# Autodesk Inventor assembly: Build Platform Assembly
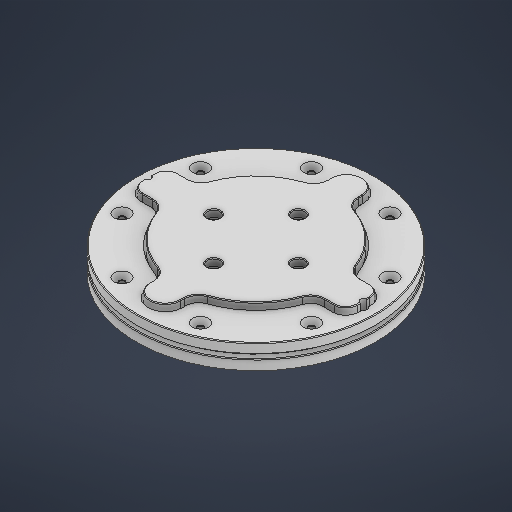
[picture p0: Inventor's stored thumbnail of the model, 512x512]
Saved by Autodesk Inventor 2025 (Build 290162000, 162)
## iProperties
Created: 2025-10-07
Part Number: Build Platform Assembly
Document SubType Name: Assembly
Designer: mayhem
Author: mayhem
## Documents named in this file (3)
- C:\Users\mayhe\OneDrive\Documents\GitHub\In-situ-monitoring-of-powder-bed-fusion-additive-manufacturing\accessories\Build platform\Build Platform Assembly.iam
- C:\Users\mayhe\OneDrive\Documents\GitHub\In-situ-monitoring-of-powder-bed-fusion-additive-manufacturing\accessories\Build platform\Updated Build Platform.ipt
- C:\Users\mayhe\OneDrive\Documents\GitHub\In-situ-monitoring-of-powder-bed-fusion-additive-manufacturing\accessories\Build platform\Clamp Ring.ipt
## Components (2 placed, 2 different names)
1. Updated Build Platform:1 — Rotational:1
2. Clamp Ring:2 — Rotational:1
## Relationships (1: RevoluteJoint 1)
- Rotational:1 [RevoluteJoint]: Updated Build Platform:1 ↔ Clamp Ring:2
